# Autodesk Inventor assembly: 8 ball mechanism
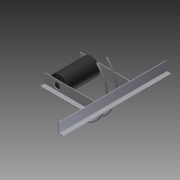
[picture p0: Inventor's stored thumbnail of the model, 180x180]
Saved by Autodesk Inventor 2012 (Build 160160000, 160)
## iProperties
Created: 2013-09-05
Part Number: 8 ball mechanism
Document SubType Name: Assembly
Designer: Bryce
Author: Bryce
## Documents named in this file (7)
- C:\Users\Bryce\Dropbox\Inventor Design Project Files\Independent Swerves\Inventor 2012\8 ball mechanism.iam
- C:\Users\Bryce\Dropbox\Inventor Design Project Files\Independent Swerves\Inventor 2012\1 by 3 U.ipt
- C:\Users\Bryce\Dropbox\Inventor Design Project Files\Independent Swerves\Inventor 2012\8 ball bearing plate left.ipt
- C:\Users\Bryce\Dropbox\Inventor Design Project Files\Independent Swerves\Inventor 2012\8 ball bearing plate right.ipt
- C:\Users\Bryce\Dropbox\Inventor Design Project Files\Independent Swerves\Inventor 2012\8 ball roller.ipt
- C:\Users\Bryce\Dropbox\Inventor Design Project Files\Independent Swerves\Inventor 2012\8 ball L frame.ipt
- C:\Users\Bryce\Dropbox\Inventor Design Project Files\Independent Swerves\Inventor 2012\8 ball arch.ipt
## Components (7 placed, 6 different names)
1. 1 by 3 U:1 — Mate:1, Mate:2, Flush:1, Mate:3, Mate:4, Flush:2
2. 8 ball bearing plate left:1 — Mate:1, Mate:2, Flush:1
3. 8 ball bearing plate right:1 — Mate:3, Mate:4, Flush:2, Mate:5, Mate:6, Mate:7, Flush:3, Flush:4
4. 8 ball roller:1 — Mate:5, Mate:6, Mate:8, Mate:9
5. 8 ball L frame:1 — Mate:7, Flush:3, Flush:4
6. 8 ball arch:1 — Mate:9
7. 8 ball arch:2 — Mate:8
## Relationships (13: Mate 9, Flush 4)
- Mate:1: 1 by 3 U:1 ↔ 8 ball bearing plate left:1
- Mate:2: 1 by 3 U:1 ↔ 8 ball bearing plate left:1
- Flush:1: 1 by 3 U:1 ↔ 8 ball bearing plate left:1
- Mate:3: 1 by 3 U:1 ↔ 8 ball bearing plate right:1
- Mate:4: 1 by 3 U:1 ↔ 8 ball bearing plate right:1
- Flush:2: 1 by 3 U:1 ↔ 8 ball bearing plate right:1
- Mate:5: 8 ball bearing plate right:1 ↔ 8 ball roller:1
- Mate:6 (6.35 mm): 8 ball bearing plate right:1 ↔ 8 ball roller:1
- Mate:7: 8 ball bearing plate right:1 ↔ 8 ball L frame:1
- Flush:3: 8 ball bearing plate right:1 ↔ 8 ball L frame:1
- Flush:4 (184.15 mm): 8 ball bearing plate right:1 ↔ 8 ball L frame:1
- Mate:8: 8 ball roller:1 ↔ 8 ball arch:2
- Mate:9: 8 ball roller:1 ↔ 8 ball arch:1
